# Autodesk Inventor assembly: Knobber
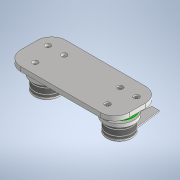
[picture p0: Inventor's stored thumbnail of the model, 180x180]
Saved by Autodesk Inventor 2021 (Build 250183000, 183)
## iProperties
Created: 2024-03-24
Part Number: Knobber
Document SubType Name: Assembly
Designer: Lukas
Author: Lukas
## Documents named in this file (9)
- \\192.168.1.200\Storragepool\Datastorrage\Projects\Knobber\Mechanics\Knobber.iam
- \\192.168.1.200\Storragepool\Datastorrage\Projects\Knobber\Mechanics\XXX.XXXXPCB_Assy_Revision_Knobber.iam
- \\192.168.1.200\Storragepool\Datastorrage\Projects\Knobber\Mechanics\ML2204B 2204-260kv.ipt
- \\192.168.1.200\Storragepool\Datastorrage\Projects\Knobber\Mechanics\Spacerplate.ipt
- \\192.168.1.200\Storragepool\Datastorrage\Projects\Knobber\Mechanics\Baseplate.ipt
- \\192.168.1.200\Storragepool\Datastorrage\Projects\Knobber\Mechanics\M3x12.ipt
- \\192.168.1.200\Storragepool\Datastorrage\Projects\Knobber\Mechanics\M2x4.ipt
- \\192.168.1.200\Storragepool\Datastorrage\Projects\Knobber\Mechanics\Magnethalter.ipt
- \\192.168.1.200\Storragepool\Datastorrage\Projects\Knobber\Mechanics\Pointerlever.ipt
## Components (22 placed, 8 different names)
1. Baseplate:1 — Mate:11, Mate:12, Mate:13, Insert:13, Insert:14, Insert:15, Mate:17, Mate:18, Mate:19
2. XXX.XXXXPCB_Assy_Revision_Knobber:1 [sub-assembly] — Mate:1, Flush:1, Flush:2, Flush:3, Mate:2, Mate:3, Mate:4, Mate:11, Mate:12, Mate:13
3. XXX.XXXXPCB_Assy_Revision_Knobber:2 [sub-assembly] — Mate:17, Mate:18, Mate:19, Mate:20, Mate:21, Mate:22
4. ML2204B 2204-260kv:1 — Mate:1, Angle:1, Mate:10, Insert:12, Angle:14, Mate:14, Mate:16, Flush:4
5. ML2204B 2204-260kv:2 — Mate:23, Mate:24, Mate:25, Insert:20, Mate:26, Mate:27, Flush:5
6. Spacerplate:1 — Mate:2, Mate:3, Mate:4, Insert:4, Insert:5, Insert:6, Insert:7, Mate:10
7. Spacerplate:2 — Mate:20, Mate:21, Mate:22, Mate:23, Mate:24, Mate:25
8. Magnethalter:1 — Insert:12, Angle:14, Angle:19
9. Pointerlever:1 — Mate:14, Mate:16, Flush:4, Insert:16, Insert:17, Insert:18, Insert:19, Angle:18
10. Magnethalter:2 — Insert:20, Angle:19
11. Pointerlever:2 — Mate:26, Mate:27, Flush:5
12. M3x12:1 — Angle:7, Angle:8, Insert:15
13. M3x12:2 — Angle:6, Angle:7, Insert:14
14. M3x12:3 — Angle:5, Angle:6, Insert:13
15. M2x4:1 — Insert:4, Angle:4, Angle:5
16. M2x4:2 — Insert:5, Angle:3, Angle:4
17. M2x4:3 — Insert:6, Angle:2, Angle:3
18. M2x4:4 — Insert:7, Angle:2
19. M2x4:5 — Angle:12, Insert:19, Angle:16, Angle:17
20. M2x4:6 — Angle:11, Angle:12, Insert:17, Angle:15
21. M2x4:7 — Angle:10, Angle:11, Insert:18, Angle:15, Angle:16
22. M2x4:8 — Angle:10, Insert:16, Angle:17, Angle:18
## Relationships (56: Mate 21, Angle 17, Insert 13, Flush 5)
- Mate:1: XXX.XXXXPCB_Assy_Revision_Knobber:1 ↔ ML2204B 2204-260kv:1
- Flush:1: XXX.XXXXPCB_Assy_Revision_Knobber:1
- Flush:2: XXX.XXXXPCB_Assy_Revision_Knobber:1
- Flush:3: XXX.XXXXPCB_Assy_Revision_Knobber:1
- Angle:1 (-90 deg): ML2204B 2204-260kv:1
- Mate:2: XXX.XXXXPCB_Assy_Revision_Knobber:1 ↔ Spacerplate:1
- Mate:3: XXX.XXXXPCB_Assy_Revision_Knobber:1 ↔ Spacerplate:1
- Mate:4: XXX.XXXXPCB_Assy_Revision_Knobber:1 ↔ Spacerplate:1
- Insert:4: Spacerplate:1 ↔ M2x4:1
- Insert:5: Spacerplate:1 ↔ M2x4:2
- Insert:6: Spacerplate:1 ↔ M2x4:3
- Insert:7: Spacerplate:1 ↔ M2x4:4
- Angle:2 (0 deg): M2x4:3 ↔ M2x4:4
- Angle:3 (0 deg): M2x4:2 ↔ M2x4:3
- Angle:4 (0 deg): M2x4:1 ↔ M2x4:2
- Angle:5 (0 deg): M3x12:3 ↔ M2x4:1
- Angle:6 (0 deg): M3x12:2 ↔ M3x12:3
- Angle:7 (0 deg): M3x12:1 ↔ M3x12:2
- Angle:8 (0 deg): M3x12:1
- Mate:10: ML2204B 2204-260kv:1 ↔ Spacerplate:1
- Angle:10 (0 deg): M2x4:7 ↔ M2x4:8
- Angle:11 (0 deg): M2x4:6 ↔ M2x4:7
- Angle:12 (0 deg): M2x4:5 ↔ M2x4:6
- Insert:12: ML2204B 2204-260kv:1 ↔ Magnethalter:1
- Angle:14 (0 deg): ML2204B 2204-260kv:1 ↔ Magnethalter:1
- Mate:11: Baseplate:1 ↔ XXX.XXXXPCB_Assy_Revision_Knobber:1
- Mate:12: Baseplate:1 ↔ XXX.XXXXPCB_Assy_Revision_Knobber:1
- Mate:13: Baseplate:1 ↔ XXX.XXXXPCB_Assy_Revision_Knobber:1
- Insert:13: Baseplate:1 ↔ M3x12:3
- Insert:14: Baseplate:1 ↔ M3x12:2
- Insert:15: Baseplate:1 ↔ M3x12:1
- Mate:14: ML2204B 2204-260kv:1 ↔ Pointerlever:1
- Mate:16: ML2204B 2204-260kv:1 ↔ Pointerlever:1
- Flush:4: ML2204B 2204-260kv:1 ↔ Pointerlever:1
- Insert:16: Pointerlever:1 ↔ M2x4:8
- Insert:17: Pointerlever:1 ↔ M2x4:6
- Insert:18: Pointerlever:1 ↔ M2x4:7
- Insert:19: Pointerlever:1 ↔ M2x4:5
- Angle:15 (0 deg): M2x4:6 ↔ M2x4:7
- Angle:16 (0 deg): M2x4:5 ↔ M2x4:7
- Angle:17 (0 deg): M2x4:5 ↔ M2x4:8
- Angle:18 (0 deg): Pointerlever:1 ↔ M2x4:8
- Mate:17: Baseplate:1 ↔ XXX.XXXXPCB_Assy_Revision_Knobber:2
- Mate:18: Baseplate:1 ↔ XXX.XXXXPCB_Assy_Revision_Knobber:2
- Mate:19: Baseplate:1 ↔ XXX.XXXXPCB_Assy_Revision_Knobber:2
- Mate:20: XXX.XXXXPCB_Assy_Revision_Knobber:2 ↔ Spacerplate:2
- Mate:21: XXX.XXXXPCB_Assy_Revision_Knobber:2 ↔ Spacerplate:2
- Mate:22: XXX.XXXXPCB_Assy_Revision_Knobber:2 ↔ Spacerplate:2
- Mate:23: ML2204B 2204-260kv:2 ↔ Spacerplate:2
- Mate:24: ML2204B 2204-260kv:2 ↔ Spacerplate:2
- Mate:25: ML2204B 2204-260kv:2 ↔ Spacerplate:2
- Insert:20: ML2204B 2204-260kv:2 ↔ Magnethalter:2
- Angle:19 (0 deg): Magnethalter:1 ↔ Magnethalter:2
- Mate:26: ML2204B 2204-260kv:2 ↔ Pointerlever:2
- Mate:27: ML2204B 2204-260kv:2 ↔ Pointerlever:2
- Flush:5: ML2204B 2204-260kv:2 ↔ Pointerlever:2
